# Autodesk Inventor assembly: IntakeFilter
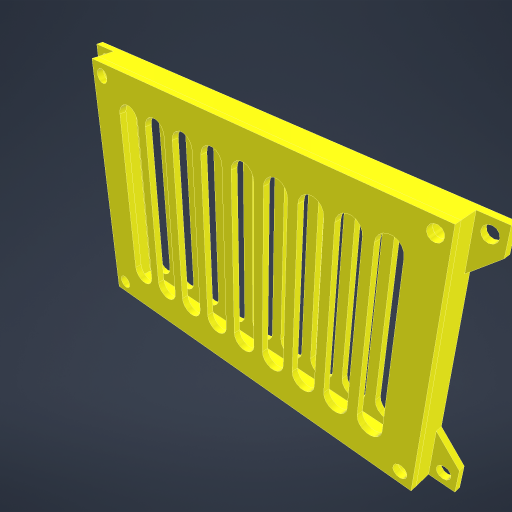
[picture p0: Inventor's stored thumbnail of the model, 512x512]
Saved by Autodesk Inventor 2024.2 (Build 282272000, 272)
## iProperties
Created: 2024-06-05
Part Number: IntakeFilter
Document SubType Name: Assembly
Designer: simon
Author: simon
## Documents named in this file (3)
- C:\Users\simon\Documents\Repositories\GrowBox\hardware\IntakeFilter\IntakeFilter.iam
- C:\Users\simon\Documents\Repositories\GrowBox\hardware\IntakeFilter\IntakeFilterTop.ipt
- C:\Users\simon\Documents\Repositories\GrowBox\hardware\IntakeFilter\IntakeFilterBottom.ipt
## Components (2 placed, 2 different names)
1. IntakeFilterTop:1 — Mate:1, Mate:2, Flush:1, Flush:2, Flush:3, Mate:3
2. IntakeFilterBottom:1 — Flush:2, Flush:3, Mate:3
## Relationships (6: Mate 3, Flush 3)
- Mate:1: IntakeFilterTop:1
- Mate:2: IntakeFilterTop:1
- Flush:1: IntakeFilterTop:1
- Flush:2: IntakeFilterTop:1 ↔ IntakeFilterBottom:1
- Flush:3: IntakeFilterTop:1 ↔ IntakeFilterBottom:1
- Mate:3: IntakeFilterTop:1 ↔ IntakeFilterBottom:1
